# Autodesk Inventor assembly: V4Climb
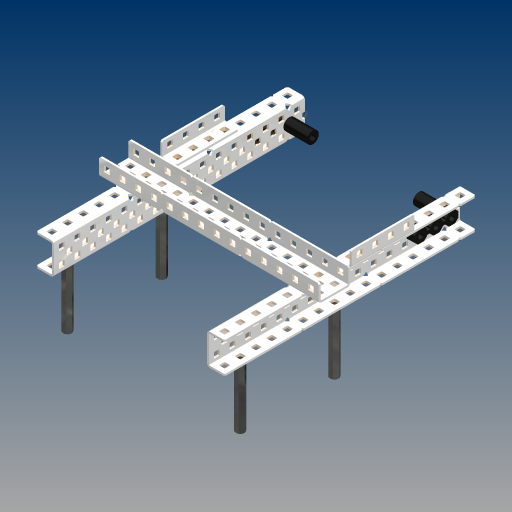
[picture p0: Inventor's stored thumbnail of the model, 512x512]
Saved by Autodesk Inventor 2023 (Build 270158000, 158)
## iProperties
Created: 2024-02-02
Part Number: V4Climb
Document SubType Name: Assembly
Designer: eddie
Author: eddie
## Documents named in this file (10)
- C:\Users\eddie\Documents\81208X-Over-Under-CAD\V4\V4Climb.iam
- C:\Users\eddie\Documents\81208X-Over-Under-CAD\VEX-CAD-Inventor-1.4.0\Structure\C Channel\Aluminum 1x2x1\Alu C 1x2x1x16.ipt
- C:\Users\eddie\Documents\81208X-Over-Under-CAD\VEX-CAD-Inventor-1.4.0\Structure\C Channel\Aluminum 1x2x1\Alu C 1x2x1x14.ipt
- C:\Users\eddie\Documents\81208X-Over-Under-CAD\VEX-CAD-Inventor-1.4.0\Structure\Standoff\Standoff 2.00.ipt
- C:\Users\eddie\Documents\81208X-Over-Under-CAD\VEX-CAD-Inventor-1.4.0\Structure\Standoff.ipt
- C:\Users\eddie\Documents\81208X-Over-Under-CAD\VEX-CAD-Inventor-1.4.0\Motion\Shaft LS\Bearing Flat.ipt
- C:\Users\eddie\Documents\81208X-Over-Under-CAD\VEX-CAD-Inventor-1.4.0\Motion\Spacers\Spacer Nylon .375 OD\NSpacer .375 OD x .500.ipt
- C:\Users\eddie\Documents\81208X-Over-Under-CAD\VEX-CAD-Inventor-1.4.0\Motion\Spacers\Spacer Nylon .375 OD.ipt
- C:\Users\eddie\Documents\81208X-Over-Under-CAD\VEX-CAD-Inventor-1.4.0\Motion\Spacers\Spacer Nylon .375 OD\NSpacer .375 OD x .250.ipt
- C:\Users\eddie\Documents\81208X-Over-Under-CAD\VEX-CAD-Inventor-1.4.0\Structure\Angle\Aluminum\1x1\Alu Angle 1x1x4.ipt
## Components (15 placed, 7 different names)
1. Alu C 1x2x1x16:1 — Insert:5, Insert:6, Insert:7, Insert:9, Insert:13, Insert:15
2. Alu C 1x2x1x16:2 — Insert:3, Insert:4, Insert:8, Insert:10, Insert:14
3. Standoff 2.00:1 — Insert:5
4. Standoff 2.00:2 — Insert:3
5. Standoff 2.00:3 — Insert:4
6. Standoff 2.00:4 — Insert:6
7. Bearing Flat:1 — Insert:7
8. Bearing Flat:2 — Insert:8
9. NSpacer .375 OD x .500:1 — Insert:9, Insert:11
10. NSpacer .375 OD x .500:2 — Insert:10, Insert:12
11. NSpacer .375 OD x .250:3 — Insert:11
12. NSpacer .375 OD x .250:4 — Insert:12
13. Alu C 1x2x1x14:2 — Insert:13
14. Alu Angle 1x1x4:1 — Insert:15
15. Alu Angle 1x1x4:2 — Insert:14
## Relationships (13: Insert 13)
- Insert:3: Alu C 1x2x1x16:2 ↔ Standoff 2.00:2
- Insert:4: Alu C 1x2x1x16:2 ↔ Standoff 2.00:3
- Insert:5: Alu C 1x2x1x16:1 ↔ Standoff 2.00:1
- Insert:6: Alu C 1x2x1x16:1 ↔ Standoff 2.00:4
- Insert:7: Alu C 1x2x1x16:1 ↔ Bearing Flat:1
- Insert:8: Alu C 1x2x1x16:2 ↔ Bearing Flat:2
- Insert:9: Alu C 1x2x1x16:1 ↔ NSpacer .375 OD x .500:1
- Insert:10: Alu C 1x2x1x16:2 ↔ NSpacer .375 OD x .500:2
- Insert:11: NSpacer .375 OD x .500:1 ↔ NSpacer .375 OD x .250:3
- Insert:12: NSpacer .375 OD x .500:2 ↔ NSpacer .375 OD x .250:4
- Insert:13: Alu C 1x2x1x16:1 ↔ Alu C 1x2x1x14:2
- Insert:14: Alu C 1x2x1x16:2 ↔ Alu Angle 1x1x4:2
- Insert:15: Alu C 1x2x1x16:1 ↔ Alu Angle 1x1x4:1
